# Autodesk Inventor assembly: OdometryAssembly_MIR
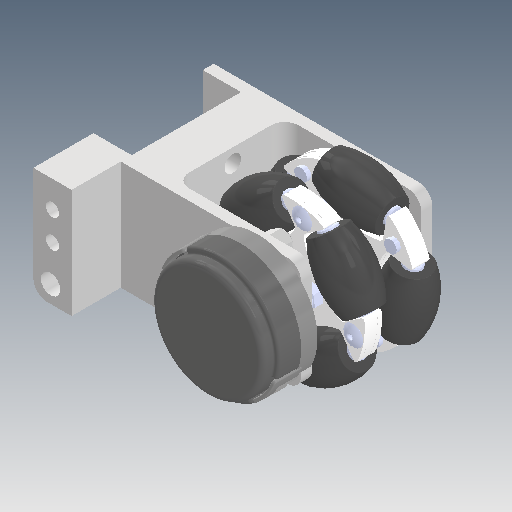
[picture p0: Inventor's stored thumbnail of the model, 512x512]
Saved by Autodesk Inventor 2020 (Build 240168000, 168)
## iProperties
Created: 2019-07-05
Part Number: OdometryAssembly_MIR
Document SubType Name: Assembly
Designer: ball
Author: ishaa
## Documents named in this file (9)
- C:\FTC\FTC8863CAD\2019 Robot\Odoemetry module\OdometryAssembly_MIR.iam
- C:\FTC\FTC8863CAD\2019 Robot\Odoemetry module\Odometry_Holder_MIR.ipt
- C:\FTC\FTC8863CAD\2019 Robot\Odoemetry module\E8T-X-236-S-D-M-X_MIR.ipt
- C:\FTC\FTC8863CAD\Actobotics\535 parts\535042_MIR.ipt
- C:\FTC\FTC8863CAD\2019 Robot\Odoemetry module\14166_MIR.iam
- C:\FTC\FTC8863CAD\2019 Robot\Odoemetry module\90576A161_MEDIUM-STRENGTH STEEL NYLON-INSERT LOCKNUT_MIR.ipt
- C:\FTC\FTC8863CAD\2019 Robot\Odoemetry module\spacerBigOdometry_MIR.ipt
- C:\FTC\FTC8863CAD\2019 Robot\Odoemetry module\spacerSmallOdometry_MIR.ipt
- C:\FTC\FTC8863CAD\Actobotics\634 parts\634064_MIR.ipt
## Components (10 placed, 8 different names)
1. Odometry_Holder_MIR:1 — Mate:1, Insert:1, Insert:2, Insert:3, Flush:1
2. E8T-X-236-S-D-M-X_MIR:1 — Mate:1, Insert:1
3. 535042_MIR:1 — Insert:2
4. 535042_MIR:2 — Insert:3, Insert:7, Mate:4
5. 14166_MIR:1 [sub-assembly]
6. 90576A161_MEDIUM-STRENGTH STEEL NYLON-INSERT LOCKNUT_MIR:1
7. 90576A161_MEDIUM-STRENGTH STEEL NYLON-INSERT LOCKNUT_MIR:2
8. spacerBigOdometry_MIR:1
9. spacerSmallOdometry_MIR:1 — Insert:7
10. 634064_MIR:1 — Flush:1, Mate:4
## Relationships (7: Insert 4, Mate 2, Flush 1)
- Mate:1: Odometry_Holder_MIR:1 ↔ E8T-X-236-S-D-M-X_MIR:1
- Insert:1: Odometry_Holder_MIR:1 ↔ E8T-X-236-S-D-M-X_MIR:1
- Insert:2: Odometry_Holder_MIR:1 ↔ 535042_MIR:1
- Insert:3: Odometry_Holder_MIR:1 ↔ 535042_MIR:2
- Insert:7: 535042_MIR:2 ↔ spacerSmallOdometry_MIR:1
- Flush:1: Odometry_Holder_MIR:1 ↔ 634064_MIR:1
- Mate:4: 535042_MIR:2 ↔ 634064_MIR:1
